# Autodesk Inventor assembly: Banebots RS-775 to P60 Gearbox
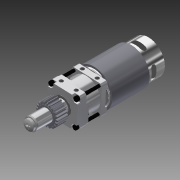
[picture p0: Inventor's stored thumbnail of the model, 180x180]
Saved by Autodesk Inventor 2014 SP1 (Build 180222100, 222)
## iProperties
Created: 2012-01-14
Part Number: Banebots RS-775 to P60 Gearbox
Document SubType Name: Assembly
Designer: Moses
Mass: 477.572 g
Surface Area: 461.809 cm^2
Volume: 64.1568 cm^3
Density: 7.44382 g/cm^3
Author: Moses
## Documents named in this file (10)
- C:\Users\Moses\Documents\GitHub\frc2014CAD\2012\Repackaged_Team_3061_Yr2012_Ball_Shooter\Banebots RS-775 to P60 Gearbox.iam
- C:\Users\Moses\Documents\GitHub\frc2014CAD\2012\Repackaged_Team_3061_Yr2012_Ball_Shooter\Motors_BaneBots_RS-775.ipt
- C:\Users\Moses\Documents\GitHub\frc2014CAD\2012\Repackaged_Team_3061_Yr2012_Ball_Shooter\AM-0129 Small Final Gear 20T.ipt
- C:\Users\Moses\Documents\GitHub\frc2014CAD\2012\Repackaged_Team_3061_Yr2012_Ball_Shooter\Aluminum Shaft Spacer P1.ipt
- C:\Users\Moses\Documents\GitHub\frc2014CAD\2012\Repackaged_Team_3061_Yr2012_Ball_Shooter\Aluminum Shaft Spacer P2.ipt
- C:\Users\Moses\Documents\GitHub\frc2014CAD\2012\Repackaged_Team_3061_Yr2012_Ball_Shooter\ASTM F436 - 1_4(1).ipt
- C:\Users\Moses\Documents\GitHub\frc2014CAD\2012\Repackaged_Team_3061_Yr2012_Ball_Shooter\ANSI B18.6.3 - 1_4-20 UNC - 0.375(14).ipt
- C:\Users\Moses\Documents\GitHub\frc2014CAD\2012\Repackaged_Team_3061_Yr2012_Ball_Shooter\Banebots RS-775 P60 Planetary Gearbox 1-Stage (0.5x1.5 shaft).iam
- C:\Users\Moses\Documents\GitHub\frc2014CAD\2012\Repackaged_Team_3061_Yr2012_Ball_Shooter\15T Gear P60 Pinion Gear.ipt
- C:\Users\Moses\Documents\GitHub\frc2014CAD\2012\Repackaged_Team_3061_Yr2012_Ball_Shooter\0.125 x 0.125 x 0.57 Key.ipt
## Components (9 placed, 9 different names)
1. Motors_BaneBots_RS-775:1 — Mate:5, Mate:6, Mate:7, Mate:8, Mate:9, Mate:10
2. AM-0129 Small Final Gear 20T:1 — Mate:4, Mate:12, Mate:13, Mate:14, Mate:15, Flush:1
3. Aluminum Shaft Spacer P1:1 — Mate:4, Mate:11
4. Aluminum Shaft Spacer P2:1 — Insert:6, Mate:12
5. Circular Washer (Inch) 1/4:1 — Insert:4, Insert:5, Insert:6
6. Cross Recessed Binding Head Machine Screw - Type I - Inch 1/4 - 20 - 3/8:1 — Insert:4
7. Banebots RS-775 P60 Planetary Gearbox 1-Stage (0.5x1.5 shaft):1 [sub-assembly] — Mate:7, Mate:8, Mate:9, Mate:10, Insert:5, Mate:11, Mate:13, Mate:14, Mate:15, Mate:16, Mate:17, Rotation:1
8. 15T Gear P60 Pinion Gear:1 — Mate:5, Mate:6, Rotation:1
9. 0.125 x 0.125 x 0.57 Key:1 — Mate:16, Mate:17, Flush:1
## Relationships (19: Mate 14, Insert 3, Flush 1, RelateRotation 1)
- Mate:4: AM-0129 Small Final Gear 20T:1 ↔ Aluminum Shaft Spacer P1:1
- Insert:4: Circular Washer (Inch) 1/4:1 ↔ Cross Recessed Binding Head Machine Screw - Type I - Inch 1/4 - 20 - 3/8:1
- Mate:5: Motors_BaneBots_RS-775:1 ↔ 15T Gear P60 Pinion Gear:1
- Mate:6 (0.5 mm): Motors_BaneBots_RS-775:1 ↔ 15T Gear P60 Pinion Gear:1
- Mate:7: Motors_BaneBots_RS-775:1 ↔ Banebots RS-775 P60 Planetary Gearbox 1-Stage (0.5x1.5 shaft):1
- Mate:8: Motors_BaneBots_RS-775:1 ↔ Banebots RS-775 P60 Planetary Gearbox 1-Stage (0.5x1.5 shaft):1
- Mate:9: Motors_BaneBots_RS-775:1 ↔ Banebots RS-775 P60 Planetary Gearbox 1-Stage (0.5x1.5 shaft):1
- Mate:10: Motors_BaneBots_RS-775:1 ↔ Banebots RS-775 P60 Planetary Gearbox 1-Stage (0.5x1.5 shaft):1
- Insert:5: Circular Washer (Inch) 1/4:1 ↔ Banebots RS-775 P60 Planetary Gearbox 1-Stage (0.5x1.5 shaft):1
- Insert:6: Aluminum Shaft Spacer P2:1 ↔ Circular Washer (Inch) 1/4:1
- Mate:11: Aluminum Shaft Spacer P1:1 ↔ Banebots RS-775 P60 Planetary Gearbox 1-Stage (0.5x1.5 shaft):1
- Mate:12: AM-0129 Small Final Gear 20T:1 ↔ Aluminum Shaft Spacer P2:1
- Mate:13: AM-0129 Small Final Gear 20T:1 ↔ Banebots RS-775 P60 Planetary Gearbox 1-Stage (0.5x1.5 shaft):1
- Mate:14: AM-0129 Small Final Gear 20T:1 ↔ Banebots RS-775 P60 Planetary Gearbox 1-Stage (0.5x1.5 shaft):1
- Mate:15: AM-0129 Small Final Gear 20T:1 ↔ Banebots RS-775 P60 Planetary Gearbox 1-Stage (0.5x1.5 shaft):1
- Mate:16: Banebots RS-775 P60 Planetary Gearbox 1-Stage (0.5x1.5 shaft):1 ↔ 0.125 x 0.125 x 0.57 Key:1
- Mate:17: Banebots RS-775 P60 Planetary Gearbox 1-Stage (0.5x1.5 shaft):1 ↔ 0.125 x 0.125 x 0.57 Key:1
- Flush:1: AM-0129 Small Final Gear 20T:1 ↔ 0.125 x 0.125 x 0.57 Key:1
- Rotation:1 [RelateRotation] (4 ul): Banebots RS-775 P60 Planetary Gearbox 1-Stage (0.5x1.5 shaft):1 ↔ 15T Gear P60 Pinion Gear:1
